# Autodesk Inventor assembly: Assembly111
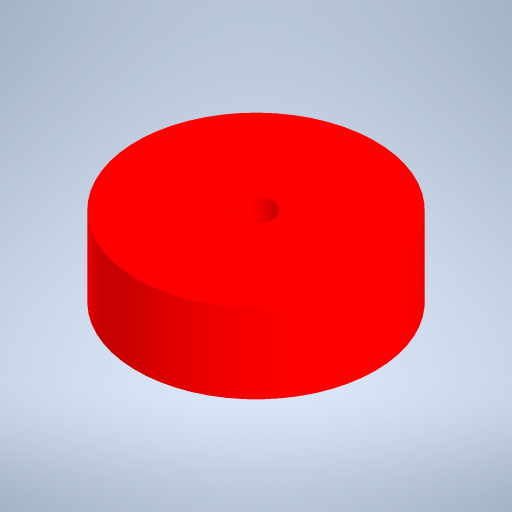
[picture p0: Inventor's stored thumbnail of the model, 512x512]
Saved by Autodesk Inventor 2023 (Build 270158000, 158)
## iProperties
Created: 2023-01-31
Part Number: Assembly111
Document SubType Name: Assembly
Designer: Umut Yücesoy
Author: Umut Yücesoy
## Documents named in this file (3)
- C:\Users\ycsyy\Desktop\HARİKA KUMANDA TASARIMI\Assembly111.iam
- C:\Users\ycsyy\Desktop\kumandadış.ipt
- C:\Users\ycsyy\Desktop\kumandaiç.ipt
## Components (2 placed, 2 different names)
1. kumandadış:1 — Mate:1, Mate:2
2. kumandaiç:1 — Mate:1, Mate:2
## Relationships (2: Mate 2)
- Mate:1: kumandadış:1 ↔ kumandaiç:1
- Mate:2: kumandadış:1 ↔ kumandaiç:1
